# Autodesk Inventor assembly: Infill3DExtruder
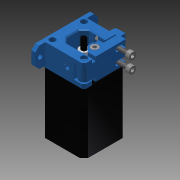
[picture p0: Inventor's stored thumbnail of the model, 180x180]
Saved by Autodesk Inventor 2015 SP1 (Build 190203100, 203)
## iProperties
Created: 2015-04-27
Part Number: Infill3DExtruder
Document SubType Name: Assembly
Designer: Jack
Author: Jack
## Documents named in this file (9)
- C:\Users\Jack\ownCloud\Projects\CrossBot\InventorModel\Extruder\Infill3DExtruder\Infill3DExtruder.iam
- C:\Users\Jack\ownCloud\Projects\CrossBot\InventorModel\Extruder\Infill3DExtruder\Infill3DBody.ipt
- C:\Users\Jack\ownCloud\Projects\CrossBot\InventorModel\Electronics\Motors\StepperMotorNema17x60mm.ipt
- C:\Users\Jack\ownCloud\Projects\CrossBot\InventorModel\Hardware\Extruder\DriveGearMK8.ipt
- C:\Users\Jack\ownCloud\Projects\CrossBot\InventorModel\Extruder\Infill3DExtruder\Infill3DIdler.ipt
- C:\Users\Jack\ownCloud\Projects\CrossBot\InventorModel\Hardware\Bearing\BearingRadialBall\BearingRadialBall624zz.ipt
- C:\Users\Jack\ownCloud\Projects\CrossBot\InventorModel\Hardware\Nuts\Nut4.ipt
- C:\Users\Jack\ownCloud\Projects\CrossBot\InventorModel\Hardware\Bolts\SHCS\SHCS4\SHCS4x16.ipt
- C:\Users\Jack\ownCloud\Projects\CrossBot\InventorModel\Hardware\Bolts\SHCS\SHCS4\SHCS4x30.ipt
## Components (11 placed, 8 different names)
1. Infill3DBody:1 — Mate:1, Mate:2, Mate:6, Mate:7, Mate:8, Mate:15, Mate:16, Mate:18, Mate:20, Angle:2, Angle:3
2. StepperMotorNema17x60mm:1 — Mate:1, Mate:2, Mate:4, Mate:5, Mate:6
3. DriveGearMK8:1 — Mate:4, Mate:5
4. Infill3DIdler:1 — Mate:7, Mate:8, Mate:9, Mate:10, Mate:11, Mate:12, Angle:1, Mate:13, Mate:14
5. BearingRadialBall624zz:1 — Mate:9, Mate:10
6. Nut4:1 — Mate:11, Mate:12, Angle:1
7. SHCS4x16:1 — Mate:13, Mate:14
8. SHCS4x30:1 — Mate:15, Mate:17, Flush:1
9. SHCS4x30:2 — Mate:16, Mate:19, Flush:1
10. Nut4:2 — Mate:17, Mate:18, Angle:3
11. Nut4:3 — Mate:19, Mate:20, Angle:2
## Relationships (23: Mate 19, Angle 3, Flush 1)
- Mate:1: Infill3DBody:1 ↔ StepperMotorNema17x60mm:1
- Mate:2: Infill3DBody:1 ↔ StepperMotorNema17x60mm:1
- Mate:4: StepperMotorNema17x60mm:1 ↔ DriveGearMK8:1
- Mate:5 (1 mm): StepperMotorNema17x60mm:1 ↔ DriveGearMK8:1
- Mate:6: Infill3DBody:1 ↔ StepperMotorNema17x60mm:1
- Mate:7: Infill3DBody:1 ↔ Infill3DIdler:1
- Mate:8 (0.2 mm): Infill3DBody:1 ↔ Infill3DIdler:1
- Mate:9: Infill3DIdler:1 ↔ BearingRadialBall624zz:1
- Mate:10: Infill3DIdler:1 ↔ BearingRadialBall624zz:1
- Mate:11: Infill3DIdler:1 ↔ Nut4:1
- Mate:12: Infill3DIdler:1 ↔ Nut4:1
- Angle:1 (0 deg): Infill3DIdler:1 ↔ Nut4:1
- Mate:13: Infill3DIdler:1 ↔ SHCS4x16:1
- Mate:14: Infill3DIdler:1 ↔ SHCS4x16:1
- Mate:15: Infill3DBody:1 ↔ SHCS4x30:1
- Mate:16: Infill3DBody:1 ↔ SHCS4x30:2
- Mate:17: SHCS4x30:1 ↔ Nut4:2
- Mate:18: Infill3DBody:1 ↔ Nut4:2
- Mate:19: SHCS4x30:2 ↔ Nut4:3
- Mate:20: Infill3DBody:1 ↔ Nut4:3
- Angle:2 (0 deg): Infill3DBody:1 ↔ Nut4:3
- Angle:3 (0 deg): Infill3DBody:1 ↔ Nut4:2
- Flush:1: SHCS4x30:1 ↔ SHCS4x30:2
